# Autodesk Inventor assembly: arm_himo
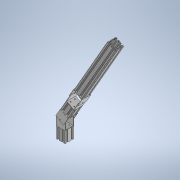
[picture p0: Inventor's stored thumbnail of the model, 180x180]
Saved by Autodesk Inventor 2021.4 (Build 254397000, 397)
## iProperties
Created: 2023-10-13
Part Number: arm_himo
Document SubType Name: Assembly
Designer: ryusei
Author: ryusei
## Documents named in this file (5)
- G:\マイドライブ\千葉工業大学\RDC Lab\引き紐（人追従）\ハードウェア\引き紐\arm_himo.iam
- G:\マイドライブ\千葉工業大学\RDC Lab\引き紐（人追従）\ハードウェア\引き紐\HFS5-4040-50.ipt
- G:\マイドライブ\千葉工業大学\RDC Lab\引き紐（人追従）\ハードウェア\引き紐\blaket_1.ipt
- G:\マイドライブ\千葉工業大学\RDC Lab\引き紐（人追従）\ハードウェア\引き紐\blaket_2.ipt
- G:\マイドライブ\千葉工業大学\RDC Lab\引き紐（人追従）\ハードウェア\引き紐\HFS5-4040-300.ipt
## Components (7 placed, 4 different names)
1. HFS5-4040-50:1 — 挿入:1, 挿入:2
2. HFS5-4040-50:2 — 挿入:5, 挿入:6, 挿入:7, 挿入:8, 角度:1
3. blaket_1:1 — 挿入:1, 挿入:2, 挿入:3, 挿入:4
4. blaket_1:2 — 挿入:7, 挿入:8, 挿入:9, 挿入:10
5. blaket_2:1 — 挿入:3, 挿入:4, 挿入:5, 挿入:6
6. blaket_2:2 — 挿入:9, 挿入:10, 挿入:11, 挿入:12
7. HFS5-4040-300:1 — 挿入:11, 挿入:12, 角度:1
## Relationships (13: Insert 12, Angle 1)
- 挿入:1 [Insert]: HFS5-4040-50:1 ↔ blaket_1:1
- 挿入:2 [Insert]: HFS5-4040-50:1 ↔ blaket_1:1
- 挿入:3 [Insert]: blaket_1:1 ↔ blaket_2:1
- 挿入:4 [Insert]: blaket_1:1 ↔ blaket_2:1
- 挿入:5 [Insert]: HFS5-4040-50:2 ↔ blaket_2:1
- 挿入:6 [Insert]: HFS5-4040-50:2 ↔ blaket_2:1
- 挿入:7 [Insert]: HFS5-4040-50:2 ↔ blaket_1:2
- 挿入:8 [Insert]: HFS5-4040-50:2 ↔ blaket_1:2
- 挿入:9 [Insert]: blaket_1:2 ↔ blaket_2:2
- 挿入:10 [Insert]: blaket_1:2 ↔ blaket_2:2
- 挿入:11 [Insert]: blaket_2:2 ↔ HFS5-4040-300:1
- 挿入:12 [Insert]: blaket_2:2 ↔ HFS5-4040-300:1
- 角度:1 [Angle] (0 deg): HFS5-4040-50:2 ↔ HFS5-4040-300:1
